# Autodesk Inventor assembly: Achsverbindung
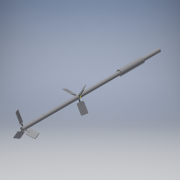
[picture p0: Inventor's stored thumbnail of the model, 180x180]
Saved by Autodesk Inventor 2017 (Build 210142000, 142)
## iProperties
Created: 2019-06-25
Part Number: Achsverbindung
Document SubType Name: Assembly
Designer: Ole Simmering
Author: Ole Simmering
## Documents named in this file (6)
- C:\Users\Ole Simmering\Documents\GitHub\3D_modeling\Konstruktion und Apparatebau\HA5-Rührreaktor\Achsverbindung.iam
- C:\Users\Ole Simmering\Documents\GitHub\3D_modeling\Konstruktion und Apparatebau\HA5-Rührreaktor\Achse.ipt
- C:\Users\Ole Simmering\Documents\GitHub\3D_modeling\Konstruktion und Apparatebau\HA5-Rührreaktor\ObererRührer.iam
- C:\Users\Ole Simmering\Documents\GitHub\3D_modeling\Konstruktion und Apparatebau\HA5-Rührreaktor\Steckhülse.ipt
- C:\Users\Ole Simmering\Documents\GitHub\3D_modeling\Konstruktion und Apparatebau\HA5-Rührreaktor\UntererRührer.iam
- C:\Users\Ole Simmering\Documents\GitHub\3D_modeling\Konstruktion und Apparatebau\HA5-Rührreaktor\Achsverbindung\Design Accelerator\Bolted Connection1.iam
## Components (7 placed, 5 different names)
1. Achse:1 — Insert:1, Angle:1, Mate:2
2. ObererRührer:1 [sub-assembly] — Insert:1, Angle:1, Insert:2, Angle:2
3. Steckhülse:1 — Insert:4, Angle:4, Insert:5, Angle:5
4. UntererRührer:1 [sub-assembly] — Insert:5, Angle:5, Mate:1
5. Steckhülse:2 — Insert:3, Angle:3, Insert:4, Angle:4
6. Steckhülse:3 — Insert:2, Angle:2, Insert:3, Angle:3
7. Bolted Connection:1 [sub-assembly] — Mate:1, Mate:2
## Relationships (12: Insert 5, Angle 5, Mate 2)
- Insert:1: Achse:1 ↔ ObererRührer:1
- Angle:1 (0 deg): Achse:1 ↔ ObererRührer:1
- Insert:2: ObererRührer:1 ↔ Steckhülse:3
- Angle:2 (0 deg): ObererRührer:1 ↔ Steckhülse:3
- Insert:3: Steckhülse:2 ↔ Steckhülse:3
- Angle:3 (0 deg): Steckhülse:2 ↔ Steckhülse:3
- Insert:4: Steckhülse:1 ↔ Steckhülse:2
- Angle:4 (0 deg): Steckhülse:1 ↔ Steckhülse:2
- Insert:5: Steckhülse:1 ↔ UntererRührer:1
- Angle:5 (0 deg): Steckhülse:1 ↔ UntererRührer:1
- Mate:1: UntererRührer:1 ↔ Bolted Connection:1
- Mate:2: Achse:1 ↔ Bolted Connection:1
